# Autodesk Inventor assembly: middle_chassis
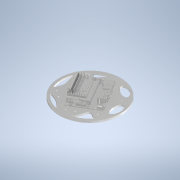
[picture p0: Inventor's stored thumbnail of the model, 180x180]
Saved by Autodesk Inventor 2020.2 (Build 242310000, 310)
## iProperties
Created: 2020-11-22
Part Number: middle_chassis
Document SubType Name: Assembly
Designer: mazzo
Author: mazzo
## Documents named in this file (3)
- D:\Documenti\università\Progetto Meccanica dei Robot\assembled in urdf\middle_chassis.iam
- D:\Documenti\università\Progetto Meccanica dei Robot\meccanica\parti autodesk\V6\V6 Luca\Jetson_Nano_DK_v1.2.ipt
- D:\Documenti\università\Progetto Meccanica dei Robot\meccanica\parti autodesk\V6\V6 Luca\middle_chassis.ipt
## Components (2 placed, 2 different names)
1. Jetson_Nano_DK_v1.2:1 — Coincidente:4, Coincidente:5, Coincidente:6
2. middle_chassis:1 — Coincidente:1, Coincidente:2, Coincidente:3, Coincidente:4, Coincidente:5, Coincidente:6
## Relationships (6: Mate 6)
- Coincidente:1 [Mate]: middle_chassis:1
- Coincidente:2 [Mate]: middle_chassis:1
- Coincidente:3 [Mate]: middle_chassis:1
- Coincidente:4 [Mate]: Jetson_Nano_DK_v1.2:1 ↔ middle_chassis:1
- Coincidente:5 [Mate]: Jetson_Nano_DK_v1.2:1 ↔ middle_chassis:1
- Coincidente:6 [Mate]: Jetson_Nano_DK_v1.2:1 ↔ middle_chassis:1
